# Autodesk Inventor assembly: MECANISMO DE COMPACTADO CON RODILLOS
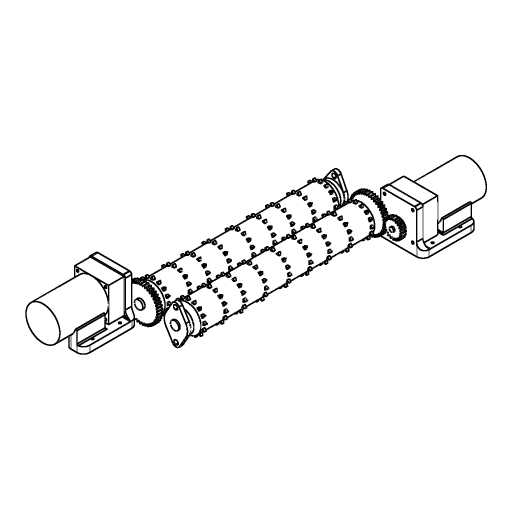
[picture p0: Inventor's stored thumbnail of the model, 512x512]
Saved by Autodesk Inventor 2024 (Build 280153000, 153)
## iProperties
Created: 2024-05-26
Part Number: MECANISMO DE COMPACTADO CON RODILLOS
Document SubType Name: Assembly
Designer: Jhuliams
Author: Jhuliams
## Documents named in this file (7)
- C:\Users\Jhuliams\Documents\GitHub\RECICLADOR_MODELO_3D\MECANISMO DE COMPACTADO\MECANISMO DE COMPACTADO CON RODILLOS.iam
- C:\Users\Jhuliams\Documents\GitHub\RECICLADOR_MODELO_3D\MECANISMO DE COMPACTADO\RODILLO.ipt
- C:\Users\Jhuliams\Documents\GitHub\RECICLADOR_MODELO_3D\MECANISMO DE COMPACTADO\MOTOR DC.ipt
- C:\Users\Jhuliams\Documents\GitHub\RECICLADOR_MODELO_3D\MECANISMO DE COMPACTADO\SOPORTE DEL MOTOR_MIR.ipt
- C:\Users\Jhuliams\Documents\GitHub\RECICLADOR_MODELO_3D\MECANISMO DE COMPACTADO\ENGRANAJE PARA RODILLO.ipt
- C:\Users\Jhuliams\Documents\GitHub\RECICLADOR_MODELO_3D\MECANISMO DE COMPACTADO\ENGRANAJE PARA RODILLO CONDUCIDO.ipt
- C:\Users\Jhuliams\Documents\GitHub\RECICLADOR_MODELO_3D\MECANISMO DE COMPACTADO\RODAMIENTO DE PARED.ipt
## Components (12 placed, 6 different names)
1. RODILLO:1 — Mate:65, Mate:67, Flush:17, Rotation:1, Mate:78, Flush:21, Mate:82, Mate:87, Flush:27
2. RODILLO:2 — Mate:66, Mate:67, Flush:17, Rotation:1, Mate:79, Flush:22, Mate:83, Mate:86, Flush:28
3. MOTOR DC:1 — Mate:74, Flush:19, Mate:75, Mate:85, Flush:26
4. MOTOR DC:2 — Mate:72, Flush:18, Mate:73, Flush:20, Mate:84, Flush:25
5. SOPORTE DEL MOTOR_MIR:1 — Mate:72, Flush:18, Mate:73, Mate:77
6. SOPORTE DEL MOTOR_MIR:2 — Mate:74, Flush:19, Mate:75, Mate:76
7. ENGRANAJE PARA RODILLO:1 — Mate:80, Mate:83, Flush:24, Mate:85, Flush:26
8. ENGRANAJE PARA RODILLO:2 — Mate:81, Mate:82, Flush:23, Mate:84, Flush:25
9. ENGRANAJE PARA RODILLO CONDUCIDO:1 — Mate:78, Flush:21, Flush:23
10. ENGRANAJE PARA RODILLO CONDUCIDO:2 — Mate:79, Flush:22, Flush:24
11. RODAMIENTO DE PARED:1 — Mate:86, Flush:28
12. RODAMIENTO DE PARED:2 — Mate:87, Flush:27
## Relationships (32: Mate 19, Flush 12, RelateRotation 1)
- Mate:65: RODILLO:1
- Mate:66: RODILLO:2
- Mate:67 (85 mm): RODILLO:1 ↔ RODILLO:2
- Flush:17: RODILLO:1 ↔ RODILLO:2
- Mate:72: MOTOR DC:2 ↔ SOPORTE DEL MOTOR_MIR:1
- Flush:18 (-2.5 mm): MOTOR DC:2 ↔ SOPORTE DEL MOTOR_MIR:1
- Mate:73: MOTOR DC:2 ↔ SOPORTE DEL MOTOR_MIR:1
- Mate:74: MOTOR DC:1 ↔ SOPORTE DEL MOTOR_MIR:2
- Flush:19 (-2.5 mm): MOTOR DC:1 ↔ SOPORTE DEL MOTOR_MIR:2
- Mate:75: MOTOR DC:1 ↔ SOPORTE DEL MOTOR_MIR:2
- Mate:76 (-42.5 mm): SOPORTE DEL MOTOR_MIR:2
- Mate:77 (-42.5 mm): SOPORTE DEL MOTOR_MIR:1
- Rotation:1 [RelateRotation] (1 ul): RODILLO:1 ↔ RODILLO:2
- Flush:20: MOTOR DC:2
- Mate:78: RODILLO:1 ↔ ENGRANAJE PARA RODILLO CONDUCIDO:1
- Flush:21 (5 mm): RODILLO:1 ↔ ENGRANAJE PARA RODILLO CONDUCIDO:1
- Mate:79: RODILLO:2 ↔ ENGRANAJE PARA RODILLO CONDUCIDO:2
- Flush:22 (5 mm): RODILLO:2 ↔ ENGRANAJE PARA RODILLO CONDUCIDO:2
- Mate:80: ENGRANAJE PARA RODILLO:1
- Mate:81: ENGRANAJE PARA RODILLO:2
- Mate:82 (60 mm): RODILLO:1 ↔ ENGRANAJE PARA RODILLO:2
- Flush:23: ENGRANAJE PARA RODILLO:2 ↔ ENGRANAJE PARA RODILLO CONDUCIDO:1
- Mate:83 (60 mm): RODILLO:2 ↔ ENGRANAJE PARA RODILLO:1
- Flush:24: ENGRANAJE PARA RODILLO:1 ↔ ENGRANAJE PARA RODILLO CONDUCIDO:2
- Mate:84: MOTOR DC:2 ↔ ENGRANAJE PARA RODILLO:2
- Flush:25 (-3 mm): MOTOR DC:2 ↔ ENGRANAJE PARA RODILLO:2
- Mate:85: MOTOR DC:1 ↔ ENGRANAJE PARA RODILLO:1
- Flush:26 (-3 mm): MOTOR DC:1 ↔ ENGRANAJE PARA RODILLO:1
- Mate:86: RODILLO:2 ↔ RODAMIENTO DE PARED:1
- Mate:87: RODILLO:1 ↔ RODAMIENTO DE PARED:2
- Flush:27 (3 mm): RODILLO:1 ↔ RODAMIENTO DE PARED:2
- Flush:28 (3 mm): RODILLO:2 ↔ RODAMIENTO DE PARED:1
